# Autodesk Inventor assembly: ASY mixer 2
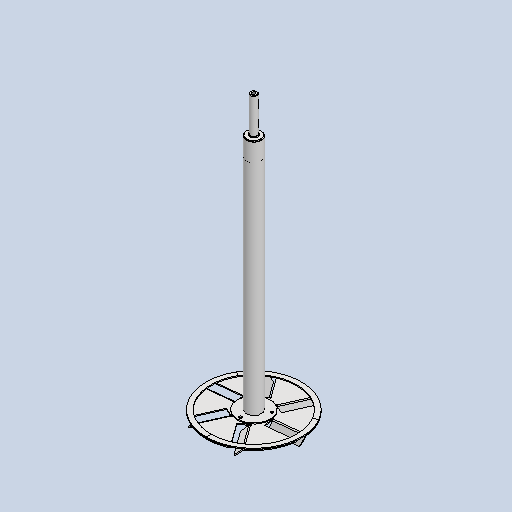
[picture p0: Inventor's stored thumbnail of the model, 512x512]
Saved by Autodesk Inventor 2025 (Build 290162010, 162A)
## iProperties
Created: 2023-08-07
Part Number: ASY mixer 2
Document SubType Name: Assembly
Designer: admin
Author: admin
## Documents named in this file (8)
- C:\Users\admin\YandexDisk-badmisterfox\домашниий пк\Inventor\BSH_Beshkino_bio_tank\3d party\Mixer 22.04.24\ASY mixer 3.iam
- C:\Users\admin\YandexDisk-badmisterfox\домашниий пк\Inventor\BSH_Beshkino_bio_tank\3d party\Mixer 22.04.24\shaft 3.ipt
- C:\Users\admin\YandexDisk-badmisterfox\домашниий пк\Inventor\BSH_Beshkino_bio_tank\3d party\Mixer 22.04.24\shaft 2.ipt
- C:\Users\admin\YandexDisk-badmisterfox\домашниий пк\Inventor\BSH_Beshkino_bio_tank\3d party\Mixer 22.04.24\втулка.ipt
- C:\Users\admin\YandexDisk-badmisterfox\домашниий пк\Inventor\BSH_Beshkino_bio_tank\3d party\Mixer 22.04.24\тарелка.ipt
- C:\Users\admin\YandexDisk-badmisterfox\домашниий пк\Inventor\BSH_Beshkino_bio_tank\3d party\Mixer 22.04.24\треть-кольцо.ipt
- C:\Users\admin\YandexDisk-badmisterfox\домашниий пк\Inventor\BSH_Beshkino_bio_tank\3d party\Mixer 22.04.24\платик крепежный.ipt
- C:\Users\admin\YandexDisk-badmisterfox\домашниий пк\Inventor\BSH_Beshkino_bio_tank\3d party\Mixer 22.04.24\Параметры.ipt
## Components (9 placed, 7 different names)
1. shaft 3:1 — Rotational:1, Rotational:5, Mate:1, Mate:2
2. shaft 2:1 — Rotational:2
3. втулка:1 — Rotational:1, Rotational:2
4. тарелка:1 — Insert:1, Mate:1
5. платик крепежный:1 — Rotational:5, Insert:1, Mate:2
6. треть-кольцо:1 — Rigid:6, Rigid:7
7. треть-кольцо:2 — Rigid:7
8. треть-кольцо:3 — Rigid:6
9. Параметры:1
## Relationships (8: RevoluteJoint 3, WeldJoint 2, Mate 2, Insert 1)
- Rotational:1 [RevoluteJoint] (-2 mm): shaft 3:1 ↔ втулка:1
- Rotational:2 [RevoluteJoint]: shaft 2:1 ↔ втулка:1
- Rotational:5 [RevoluteJoint]: shaft 3:1 ↔ платик крепежный:1
- Rigid:6 [WeldJoint]: треть-кольцо:1 ↔ треть-кольцо:3
- Rigid:7 [WeldJoint]: треть-кольцо:1 ↔ треть-кольцо:2
- Insert:1: тарелка:1 ↔ платик крепежный:1
- Mate:1: shaft 3:1 ↔ тарелка:1
- Mate:2: shaft 3:1 ↔ платик крепежный:1
